# Autodesk Inventor assembly: boe-bot
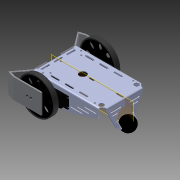
[picture p0: Inventor's stored thumbnail of the model, 180x180]
Saved by Autodesk Inventor 2015 (Build 190159000, 159)
## iProperties
Created: 2015-04-21
Part Number: boe-bot
Document SubType Name: Assembly
Designer: Kyle
Author: Kyle
Sending System: SolidWorks 2013
Last Author: Branimir
## Documents named in this file (11)
- C:\Users\Kyle\Desktop\Programming\cmp-arduino-1678\CAD\sklopovi\Imported Components\boe-bot\boe-bot.iam
- C:\Users\Kyle\Desktop\Programming\cmp-arduino-1678\CAD\sklopovi\Imported Components\boe-bot\boe-bot.ipt
- C:\Users\Kyle\Desktop\Programming\cmp-arduino-1678\CAD\sklopovi\Imported Components\boe-bot\servo motor.ipt
- C:\Users\Kyle\Desktop\Programming\cmp-arduino-1678\CAD\sklopovi\Imported Components\boe-bot\caster.ipt
- C:\Users\Kyle\Desktop\Programming\cmp-arduino-1678\CAD\sklopovi\Imported Components\boe-bot\felga.ipt
- C:\Users\Kyle\Desktop\Programming\cmp-arduino-1678\CAD\sklopovi\Imported Components\boe-bot\guma.ipt
- C:\Users\Kyle\Desktop\Programming\cmp-arduino-1678\CAD\Line Tracker v3.ipt
- C:\Users\Kyle\Desktop\Programming\cmp-arduino-1678\CAD\Encoder Mount.ipt
- C:\Users\Kyle\Desktop\Programming\cmp-arduino-1678\CAD\Encoder Mount_MIR.ipt
- C:\Users\Kyle\Desktop\Programming\cmp-arduino-1678\CAD\sklopovi\Imported Components\boe-bot\felga_MIR.ipt
- C:\Users\Kyle\Desktop\Programming\cmp-arduino-1678\CAD\sklopovi\Imported Components\boe-bot\guma_MIR.ipt
## Components (12 placed, 10 different names)
1. boe-bot:1 — Mate:3, Mate:4, Mate:5, Flush:5, Symmetry:1
2. servo motor:1 — Mate:1, Flush:2, Flush:3, Symmetry:1, Flush:6
3. servo motor:2 — Mate:2, Mate:3, Mate:4, Flush:1, Flush:4, Flush:6
4. caster:1
5. felga:3
6. guma:3
7. Line Tracker v3:1 — Mate:1, Flush:2, Flush:3
8. Line Tracker v3:2 — Mate:2, Flush:1, Flush:4
9. Encoder Mount:2 — Mate:5, Flush:5
10. Encoder Mount_MIR:1
11. felga_MIR:1
12. guma_MIR:1
## Relationships (12: Flush 6, Mate 5, Symmetry 1)
- Mate:1: servo motor:1 ↔ Line Tracker v3:1
- Mate:2: servo motor:2 ↔ Line Tracker v3:2
- Mate:3: boe-bot:1 ↔ servo motor:2
- Mate:4: boe-bot:1 ↔ servo motor:2
- Flush:1: servo motor:2 ↔ Line Tracker v3:2
- Flush:2: servo motor:1 ↔ Line Tracker v3:1
- Flush:3: servo motor:1 ↔ Line Tracker v3:1
- Flush:4: servo motor:2 ↔ Line Tracker v3:2
- Mate:5: boe-bot:1 ↔ Encoder Mount:2
- Flush:5: boe-bot:1 ↔ Encoder Mount:2
- Symmetry:1: boe-bot:1 ↔ servo motor:1
- Flush:6: servo motor:1 ↔ servo motor:2
